# Autodesk Inventor assembly: BridgeLoweringDeviceAssembly
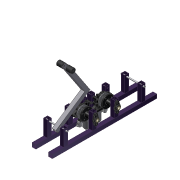
[picture p0: Inventor's stored thumbnail of the model, 180x180]
Saved by Autodesk Inventor 2012 (Build 160160000, 160)
## iProperties
Created: 2012-02-23
Part Number: BridgeLoweringDeviceAssembly
Document SubType Name: Assembly
Designer: JesseK
Author: JesseK
## Documents named in this file (9)
- Z:\UserData\Documents\Inventor\team1885frc\Robot2012\BridgeLoweringDevice\BridgeLoweringDeviceAssembly.iam
- Z:\UserData\Documents\Inventor\team1885frc\Robot2012\BridgeLoweringDevice\MainRail.ipt
- Z:\UserData\Documents\Inventor\team1885frc\Robot2012\BridgeLoweringDevice\VerticalRail.ipt
- Z:\UserData\Documents\Inventor\team1885frc\KOP Motors\ND Motor Right.iam
- Z:\UserData\Documents\Inventor\team1885frc\KOP Motors\ND Motor Left.iam
- Z:\UserData\Documents\Inventor\team1885frc\KOP Misc\igus bearing mount.iam
- Z:\UserData\Documents\Inventor\team1885frc\Robot2012\BridgeLoweringDevice\LoweringArm.ipt
- Z:\UserData\Documents\Inventor\team1885frc\Robot2012\Conveyor2\Conveyor_Roller_Middle.ipt
- Z:\UserData\Documents\Inventor\team1885frc\Robot2012\DriveTrain\DriveAxle.ipt
## Components (21 placed, 8 different names)
1. MainRail:1 — Mate:1, Flush:1, Mate:2, Mate:3, Mate:4, Mate:5, Mate:6, Mate:17, Mate:18, Mate:19, Mate:20
2. MainRail:2 — Mate:1, Flush:1, Mate:2, Mate:7, Mate:8, Mate:9, Mate:10, Mate:11, Mate:12, Mate:13, Mate:14, Mate:15, Mate:16, Flush:2, Flush:3, Mate:25, Mate:26, Mate:30
3. VerticalRail:1 — Mate:3, Mate:20, Mate:21, Mate:38, Mate:48
4. VerticalRail:2 — Mate:10, Mate:13, Mate:24, Mate:28
5. VerticalRail:3 — Mate:7, Mate:16, Mate:22, Flush:3
6. VerticalRail:4 — Mate:4, Mate:19, Mate:31
7. VerticalRail:5 — Mate:11, Mate:12, Mate:21, Flush:2, Mate:37
8. VerticalRail:6 — Mate:5, Mate:18, Mate:32
9. VerticalRail:7 — Mate:8, Mate:15, Mate:23, Mate:27, Mate:30
10. VerticalRail:8 — Mate:9, Mate:14, Mate:27, Mate:29, Flush:5, Mate:35
11. VerticalRail:9 — Mate:6, Mate:17, Mate:22, Mate:49
12. ND Motor Right:1 [sub-assembly] — Mate:23, Flush:5, Mate:34, Mate:35
13. ND Motor Left:1 [sub-assembly] — Mate:24, Flush:4, Mate:33, Mate:36
14. VerticalRail:10 — Mate:25, Mate:26, Mate:28, Mate:29, Flush:4, Mate:36
15. igus bearing mount:1 [sub-assembly] — Mate:31, Mate:33
16. igus bearing mount:2 [sub-assembly] — Mate:32, Mate:34
17. LoweringArm:1 — Mate:37, Mate:38, Mate:44, Mate:45, Mate:46
18. Conveyor_Roller_Middle:3 — Mate:44, Mate:47
19. Conveyor_Roller_Middle:4 — Mate:45, Mate:46, Mate:47
20. DriveAxle:1 — Mate:48
21. DriveAxle:2 — Mate:49
## Relationships (49: Mate 44, Flush 5)
- Mate:1 (82.55 mm): MainRail:1 ↔ MainRail:2
- Flush:1: MainRail:1 ↔ MainRail:2
- Mate:2: MainRail:1 ↔ MainRail:2
- Mate:3: MainRail:1 ↔ VerticalRail:1
- Mate:4: MainRail:1 ↔ VerticalRail:4
- Mate:5: MainRail:1 ↔ VerticalRail:6
- Mate:6: MainRail:1 ↔ VerticalRail:9
- Mate:7: MainRail:2 ↔ VerticalRail:3
- Mate:8: MainRail:2 ↔ VerticalRail:7
- Mate:9: MainRail:2 ↔ VerticalRail:8
- Mate:10: MainRail:2 ↔ VerticalRail:2
- Mate:11: MainRail:2 ↔ VerticalRail:5
- Mate:12: MainRail:2 ↔ VerticalRail:5
- Mate:13: MainRail:2 ↔ VerticalRail:2
- Mate:14: MainRail:2 ↔ VerticalRail:8
- Mate:15: MainRail:2 ↔ VerticalRail:7
- Mate:16: MainRail:2 ↔ VerticalRail:3
- Mate:17: MainRail:1 ↔ VerticalRail:9
- Mate:18: MainRail:1 ↔ VerticalRail:6
- Mate:19: MainRail:1 ↔ VerticalRail:4
- Mate:20: MainRail:1 ↔ VerticalRail:1
- Mate:21: VerticalRail:1 ↔ VerticalRail:5
- Mate:22: VerticalRail:3 ↔ VerticalRail:9
- Flush:2 (76.2 mm): MainRail:2 ↔ VerticalRail:5
- Flush:3 (76.2 mm): MainRail:2 ↔ VerticalRail:3
- Mate:23: VerticalRail:7 ↔ ND Motor Right:1
- Mate:24: VerticalRail:2 ↔ ND Motor Left:1
- Mate:25: MainRail:2 ↔ VerticalRail:10
- Mate:26: MainRail:2 ↔ VerticalRail:10
- Mate:27 (69.85 mm): VerticalRail:7 ↔ VerticalRail:8
- Mate:28 (69.85 mm): VerticalRail:2 ↔ VerticalRail:10
- Mate:29 (25.4 mm): VerticalRail:8 ↔ VerticalRail:10
- Mate:30 (-203.2 mm): MainRail:2 ↔ VerticalRail:7
- Flush:4 (-6.35 mm): ND Motor Left:1 ↔ VerticalRail:10
- Flush:5 (6.35 mm): VerticalRail:8 ↔ ND Motor Right:1
- Mate:31: VerticalRail:4 ↔ igus bearing mount:1
- Mate:32: VerticalRail:6 ↔ igus bearing mount:2
- Mate:33: ND Motor Left:1 ↔ igus bearing mount:1
- Mate:34: ND Motor Right:1 ↔ igus bearing mount:2
- Mate:35: VerticalRail:8 ↔ ND Motor Right:1
- Mate:36: ND Motor Left:1 ↔ VerticalRail:10
- Mate:37: VerticalRail:5 ↔ LoweringArm:1
- Mate:38 (12.7 mm): VerticalRail:1 ↔ LoweringArm:1
- Mate:44: LoweringArm:1 ↔ Conveyor_Roller_Middle:3
- Mate:45: LoweringArm:1 ↔ Conveyor_Roller_Middle:4
- Mate:46: LoweringArm:1 ↔ Conveyor_Roller_Middle:4
- Mate:47: Conveyor_Roller_Middle:3 ↔ Conveyor_Roller_Middle:4
- Mate:48: VerticalRail:1 ↔ DriveAxle:1
- Mate:49: VerticalRail:9 ↔ DriveAxle:2
